# Autodesk Inventor assembly: Assy
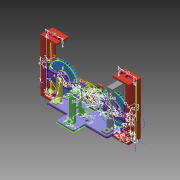
[picture p0: Inventor's stored thumbnail of the model, 180x180]
Saved by Autodesk Inventor 2014 SP1 (Build 180222100, 222)
## iProperties
Created: 2014-06-07
Part Number: Assy
Document SubType Name: Assembly
Designer: Erin
Author: Erin
## Documents named in this file (15)
- C:\Users\Erin\Desktop\AFSR\Z-axis Gantry\Assy.iam
- C:\Users\Erin\Desktop\AFSR\Z-axis Gantry\DriveGear.ipt
- C:\Users\Erin\Desktop\AFSR\Z-axis Gantry\EncoderDisk.ipt
- C:\Users\Erin\Desktop\AFSR\Z-axis Gantry\Gear1.ipt
- C:\Users\Erin\Desktop\AFSR\Z-axis Gantry\Gear2.ipt
- C:\Users\Erin\Desktop\AFSR\Z-axis Gantry\OuterBar.ipt
- C:\Users\Erin\Desktop\AFSR\Z-axis Gantry\InnerBar.ipt
- C:\Users\Erin\Desktop\AFSR\Z-axis Gantry\GearStand.ipt
- C:\Users\Erin\Desktop\AFSR\Z-axis Gantry\BottomPlate.ipt
- C:\Users\Erin\Desktop\AFSR\Z-axis Gantry\MotorMount.ipt
- C:\Users\Erin\Desktop\AFSR\Z-axis Gantry\RackSlider.ipt
- C:\Users\Erin\Desktop\AFSR\Z-axis Gantry\TopSliderBar.ipt
- C:\Users\Erin\Desktop\AFSR\Z-axis Gantry\TopSliderClip.ipt
- C:\Users\Erin\Desktop\AFSR\Z-axis Gantry\BarClip.ipt
- C:\Users\Erin\Desktop\AFSR\Z-axis Gantry\BottomSliderBar.ipt
## Components (19 placed, 13 different names)
1. Spur Gear1:1
2. EncoderDisk:1
3. Spur Gear1:2
4. Spur Gear2:1
5. Spur Gear2:2
6. OuterBar:1
7. InnerBar:1
8. GearStand:1
9. BottomPlate:1 — Insert:11
10. GearStand:2
11. MotorMount:1
12. RackSlider:2 — Insert:7, Insert:8, Insert:12
13. TopSliderBar:1 — Insert:6
14. TopSliderBar:2 — Insert:7, Insert:8, Insert:9, Insert:10
15. TopSliderClip:1 — Insert:6
16. TopSliderClip:2 — Insert:9, Insert:10
17. RackSlider:3
18. BarClip:1 — Insert:11
19. BottomSliderBar:1 — Insert:12
## Relationships (7: Insert 7)
- Insert:6: TopSliderBar:1 ↔ TopSliderClip:1
- Insert:7: RackSlider:2 ↔ TopSliderBar:2
- Insert:8: RackSlider:2 ↔ TopSliderBar:2
- Insert:9: TopSliderBar:2 ↔ TopSliderClip:2
- Insert:10: TopSliderBar:2 ↔ TopSliderClip:2
- Insert:11: BottomPlate:1 ↔ BarClip:1
- Insert:12: RackSlider:2 ↔ BottomSliderBar:1
